# Autodesk Inventor assembly: LINEAR_GUIDE_SSEB10_55_KH
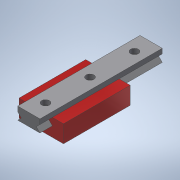
[picture p0: Inventor's stored thumbnail of the model, 180x180]
Saved by Autodesk Inventor 2020 (Build 240168000, 168)
## iProperties
Created: 2017-05-12
Part Number: LINEAR_GUIDE_SSEB10_55_KH
Material: 一般
Document SubType Name: Assembly
Designer: SHUICHI
Author: SHUICHI
## Documents named in this file (3)
- C:\Users\shun\Documents\Inventor\3wheel_omuni_2019\接地エンコーダーユニット\あ\LINEAR_GUIDE_SSEB10_55_KH.iam
- C:\Users\shun\Documents\Inventor\3wheel_omuni_2019\接地エンコーダーユニット\あ\LINEAR_GUIDE_SSEB10_KH.ipt
- C:\Users\shun\Documents\Inventor\3wheel_omuni_2019\接地エンコーダーユニット\あ\LINEAR_GUIDE_SSEB10_55_KH.ipt
## Components (2 placed, 2 different names)
1. LINEAR_GUIDE_SSEB10_KH — メイト:1, メイト:2
2. LINEAR_GUIDE_SSEB10_55_KH — メイト:1, メイト:2
## Relationships (2: Mate 2)
- メイト:1 [Mate]: LINEAR_GUIDE_SSEB10_KH ↔ LINEAR_GUIDE_SSEB10_55_KH
- メイト:2 [Mate]: LINEAR_GUIDE_SSEB10_KH ↔ LINEAR_GUIDE_SSEB10_55_KH
